# Autodesk Inventor assembly: Intake new robot
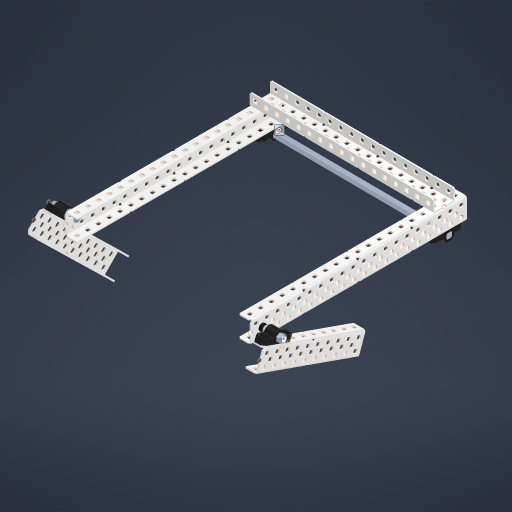
[picture p0: Inventor's stored thumbnail of the model, 512x512]
Saved by Autodesk Inventor 2023 (Build 270158000, 158)
## iProperties
Created: 2023-11-30
Part Number: Intake new robot
Document SubType Name: Assembly
Designer: diego
Author: diego
## Documents named in this file (16)
- C:\Users\diego\OneDrive\Documents\GitHub\2024-599Z\2024-599Z\Cad\Intake new robot.iam
- C:\Users\diego\OneDrive\Documents\GitHub\2024-599Z\2024-599Z\Cad\VEX-CAD-Inventor-1.4.0\Structure\C Channel\Aluminum 1x2x1\Alu C 1x2x1x20.ipt
- C:\Users\diego\OneDrive\Documents\GitHub\2024-599Z\2024-599Z\Cad\VEX-CAD-Inventor-1.4.0\Structure\Hardware\Screw Steel - Star\SScrew Star Smooth 1.000.ipt
- C:\Users\diego\OneDrive\Documents\GitHub\2024-599Z\2024-599Z\Cad\VEX-CAD-Inventor-1.4.0\Structure\Hardware\Screw Steel - Star.ipt
- C:\Users\diego\OneDrive\Documents\GitHub\2024-599Z\2024-599Z\Cad\VEX-CAD-Inventor-1.4.0\Motion\Spacers\Spacer Plastic\PSpacer 4.6.ipt
- C:\Users\diego\OneDrive\Documents\GitHub\2024-599Z\2024-599Z\Cad\VEX-CAD-Inventor-1.4.0\Motion\Spacers\Spacer Plastic.ipt
- C:\Users\diego\OneDrive\Documents\GitHub\2024-599Z\2024-599Z\Cad\VEX-CAD-Inventor-1.4.0\Structure\Hardware\Nut Keps.ipt
- C:\Users\diego\OneDrive\Documents\GitHub\2024-599Z\2024-599Z\Cad\VEX-CAD-Inventor-1.4.0\Motion\Shaft HS\HS Pillow Bearing Block.ipt
- C:\Users\diego\OneDrive\Documents\GitHub\2024-599Z\2024-599Z\Cad\VEX-CAD-Inventor-1.4.0\Structure\C Channel\Aluminum 1x2x1\Alu C 1x2x1x10.ipt
- C:\Users\diego\OneDrive\Documents\GitHub\2024-599Z\2024-599Z\Cad\VEX-CAD-Inventor-1.4.0\Structure\C Channel\Aluminum 1x2x1\Alu C 1x2x1x1.ipt
- C:\Users\diego\OneDrive\Documents\GitHub\2024-599Z\2024-599Z\Cad\VEX-CAD-Inventor-1.4.0\Structure\Hardware\Nut Nylock.ipt
- C:\Users\diego\OneDrive\Documents\GitHub\2024-599Z\2024-599Z\Cad\VEX-CAD-Inventor-1.4.0\Motion\Shaft HS\Shaft HS\Shaft HS 8.5 in.ipt
- C:\Users\diego\OneDrive\Documents\GitHub\2024-599Z\2024-599Z\Cad\VEX-CAD-Inventor-1.4.0\Motion\Shaft HS\Shaft HS.ipt
- C:\Users\diego\OneDrive\Documents\GitHub\2024-599Z\2024-599Z\Cad\VEX-CAD-Inventor-1.4.0\Motion\Shaft HS\HS Spacer\HSpacer .0625.ipt
- C:\Users\diego\OneDrive\Documents\GitHub\2024-599Z\2024-599Z\Cad\VEX-CAD-Inventor-1.4.0\Motion\Shaft HS\HS Spacer.ipt
- C:\Users\diego\OneDrive\Documents\GitHub\2024-599Z\2024-599Z\Cad\VEX-CAD-Inventor-1.4.0\Structure\C Channel\Aluminum 1x2x1\Alu C 1x2x1x17.ipt
## Components (22 placed, 11 different names)
1. Alu C 1x2x1x20:1 — Insert:8, Insert:9, Insert:17, Insert:18, Mate:11, Insert:19
2. Alu C 1x2x1x20:2 — Insert:1, Insert:2, Insert:15, Insert:16, Mate:12
3. SScrew Star Smooth 1.000:1 — Insert:8, Insert:11, Insert:12
4. SScrew Star Smooth 1.000:2 — Insert:1, Insert:4, Insert:5
5. PSpacer 4.6:1 — Insert:2, Insert:3
6. PSpacer 4.6:2 — Insert:9, Insert:10
7. Nut Keps:1 — Insert:10
8. Nut Keps:2 — Insert:3
9. HS Pillow Bearing Block:1 — Mate:3, Mate:4, Insert:13, Insert:14
10. HS Pillow Bearing Block:2 — Mate:1, Mate:2, Insert:6, Insert:7
11. Alu C 1x2x1x10:2 — Insert:6, Insert:7
12. Alu C 1x2x1x1:1 — Insert:11, Mate:3, Mate:4
13. Alu C 1x2x1x1:2 — Insert:4, Mate:1, Mate:2
14. Nut Nylock:1 — Insert:12
15. Nut Nylock:2 — Insert:5
16. Alu C 1x2x1x10:3 — Insert:13, Insert:14
17. HS Pillow Bearing Block:3 — Insert:15, Insert:16, Mate:10
18. HS Pillow Bearing Block:5 — Insert:17, Insert:18, Mate:9
19. Shaft HS 8.5 in:1 — Mate:5, Mate:6, Mate:7, Mate:8
20. HSpacer .0625:1 — Mate:5, Mate:6, Mate:9
21. HSpacer .0625:2 — Mate:7, Mate:8, Mate:10
22. Alu C 1x2x1x17:1 — Mate:11, Insert:19, Mate:12
## Relationships (31: Insert 19, Mate 12)
- Insert:1: Alu C 1x2x1x20:2 ↔ SScrew Star Smooth 1.000:2
- Insert:2: Alu C 1x2x1x20:2 ↔ PSpacer 4.6:1
- Insert:3: PSpacer 4.6:1 ↔ Nut Keps:2
- Insert:4 (-17.018 mm): SScrew Star Smooth 1.000:2 ↔ Alu C 1x2x1x1:2
- Mate:1: HS Pillow Bearing Block:2 ↔ Alu C 1x2x1x1:2
- Mate:2: HS Pillow Bearing Block:2 ↔ Alu C 1x2x1x1:2
- Insert:5 (-3.048 mm): SScrew Star Smooth 1.000:2 ↔ Nut Nylock:2
- Insert:6: HS Pillow Bearing Block:2 ↔ Alu C 1x2x1x10:2
- Insert:7: HS Pillow Bearing Block:2 ↔ Alu C 1x2x1x10:2
- Insert:8: Alu C 1x2x1x20:1 ↔ SScrew Star Smooth 1.000:1
- Insert:9: Alu C 1x2x1x20:1 ↔ PSpacer 4.6:2
- Insert:10: PSpacer 4.6:2 ↔ Nut Keps:1
- Insert:11 (-17.018 mm): SScrew Star Smooth 1.000:1 ↔ Alu C 1x2x1x1:1
- Mate:3: HS Pillow Bearing Block:1 ↔ Alu C 1x2x1x1:1
- Mate:4: HS Pillow Bearing Block:1 ↔ Alu C 1x2x1x1:1
- Insert:12 (-3.048 mm): SScrew Star Smooth 1.000:1 ↔ Nut Nylock:1
- Insert:13: HS Pillow Bearing Block:1 ↔ Alu C 1x2x1x10:3
- Insert:14: HS Pillow Bearing Block:1 ↔ Alu C 1x2x1x10:3
- Insert:15: Alu C 1x2x1x20:2 ↔ HS Pillow Bearing Block:3
- Insert:16: Alu C 1x2x1x20:2 ↔ HS Pillow Bearing Block:3
- Insert:17: Alu C 1x2x1x20:1 ↔ HS Pillow Bearing Block:5
- Insert:18: Alu C 1x2x1x20:1 ↔ HS Pillow Bearing Block:5
- Mate:5: Shaft HS 8.5 in:1 ↔ HSpacer .0625:1
- Mate:6: Shaft HS 8.5 in:1 ↔ HSpacer .0625:1
- Mate:7: Shaft HS 8.5 in:1 ↔ HSpacer .0625:2
- Mate:8: Shaft HS 8.5 in:1 ↔ HSpacer .0625:2
- Mate:9: HS Pillow Bearing Block:5 ↔ HSpacer .0625:1
- Mate:10: HS Pillow Bearing Block:3 ↔ HSpacer .0625:2
- Mate:11: Alu C 1x2x1x20:1 ↔ Alu C 1x2x1x17:1
- Insert:19: Alu C 1x2x1x20:1 ↔ Alu C 1x2x1x17:1
- Mate:12: Alu C 1x2x1x20:2 ↔ Alu C 1x2x1x17:1
